# Autodesk Inventor assembly: ChassisDes1
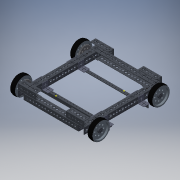
[picture p0: Inventor's stored thumbnail of the model, 180x180]
Saved by Autodesk Inventor 2016 (Build 200138000, 138)
## iProperties
Created: 2015-08-30
Part Number: ChassisDes1
Document SubType Name: Assembly
Designer: Tim
Author: Tim
## Documents named in this file (6)
- C:\Users\Tim\Documents\GitHub\phi_robotics\3d-models\FTC_Tetrix_KOP_Block_Party\Tim Bloot Designs\ChassisDes1.iam
- C:\Users\Tim\Documents\GitHub\phi_robotics\3d-models\FTC_Tetrix_KOP_Block_Party\Tim Bloot Designs\RollingSquareC1.iam
- C:\Users\Tim\Documents\GitHub\phi_robotics\3d-models\FTC_Tetrix_KOP_Block_Party\Tetrix_Kit_FTC\Autodesk Inventor Files\tetrix_corner_bracket.ipt
- C:\Users\Tim\Documents\GitHub\phi_robotics\3d-models\FTC_Tetrix_KOP_Block_Party\Tim Bloot Designs\customLbeam.ipt
- C:\Users\Tim\Documents\GitHub\phi_robotics\3d-models\FTC_Tetrix_KOP_Block_Party\Tetrix_Kit_FTC\Autodesk Inventor Files\tetrix_c_channel-4.ipt
- C:\Users\Tim\Documents\GitHub\phi_robotics\3d-models\FTC_Tetrix_KOP_Block_Party\Tetrix_Kit_FTC\Autodesk Inventor Files\tetrix_c_channel-2.ipt
## Components (18 placed, 5 different names)
1. tetrix_corner_bracket:1 — Rigid:2
2. tetrix_corner_bracket:2 — Rigid:1, Rigid:15
3. RollingSquareC1:1 [sub-assembly] — Rigid:1, Rigid:2, Rigid:16, Rigid:17, Rigid:22, Rigid:25
4. RollingSquareC1:2 [sub-assembly] — Rigid:18, Rigid:19, Rigid:23, Rigid:26
5. tetrix_corner_bracket:7 — Rigid:13
6. tetrix_corner_bracket:8
7. customLbeam:3 — Rigid:13, Rigid:15
8. customLbeam:4 — Rigid:20, Rigid:21
9. tetrix_corner_bracket:9 — Rigid:16
10. tetrix_corner_bracket:10 — Rigid:17, Rigid:20
11. tetrix_corner_bracket:11 — Rigid:19, Rigid:21
12. tetrix_corner_bracket:12 — Rigid:18
13. tetrix_c_channel-4:1 — Rigid:24
14. tetrix_c_channel-4:2 — Rotational:28
15. tetrix_c_channel-2:1 — Rigid:22, Rigid:24
16. tetrix_c_channel-2:2 — Rigid:23
17. tetrix_c_channel-2:3 — Rigid:25
18. tetrix_c_channel-2:4 — Rigid:26, Rotational:28
## Relationships (18: WeldJoint 17, RevoluteJoint 1)
- Rigid:1 [WeldJoint]: tetrix_corner_bracket:2 ↔ RollingSquareC1:1
- Rigid:2 [WeldJoint]: tetrix_corner_bracket:1 ↔ RollingSquareC1:1
- [WeldJoint]: RollingSquareC1:2 ↔ tetrix_corner_bracket:7
- [WeldJoint]: RollingSquareC1:2 ↔ tetrix_corner_bracket:8
- Rigid:13 [WeldJoint]: tetrix_corner_bracket:7 ↔ customLbeam:3
- Rigid:15 [WeldJoint]: tetrix_corner_bracket:2 ↔ customLbeam:3
- Rigid:16 [WeldJoint]: RollingSquareC1:1 ↔ tetrix_corner_bracket:9
- Rigid:17 [WeldJoint]: RollingSquareC1:1 ↔ tetrix_corner_bracket:10
- Rigid:18 [WeldJoint]: RollingSquareC1:2 ↔ tetrix_corner_bracket:12
- Rigid:19 [WeldJoint]: RollingSquareC1:2 ↔ tetrix_corner_bracket:11
- Rigid:20 [WeldJoint]: customLbeam:4 ↔ tetrix_corner_bracket:10
- Rigid:21 [WeldJoint]: customLbeam:4 ↔ tetrix_corner_bracket:11
- Rigid:22 [WeldJoint]: RollingSquareC1:1 ↔ tetrix_c_channel-2:1
- Rigid:23 [WeldJoint]: RollingSquareC1:2 ↔ tetrix_c_channel-2:2
- Rigid:24 [WeldJoint]: tetrix_c_channel-4:1 ↔ tetrix_c_channel-2:1
- Rigid:25 [WeldJoint]: RollingSquareC1:1 ↔ tetrix_c_channel-2:3
- Rigid:26 [WeldJoint]: RollingSquareC1:2 ↔ tetrix_c_channel-2:4
- Rotational:28 [RevoluteJoint]: tetrix_c_channel-4:2 ↔ tetrix_c_channel-2:4
## Named parameters: d9_d4 = 0 mm, d10_d8 = 0 mm
